# Autodesk Inventor assembly: ASSY,MK4i,Swerve_Module
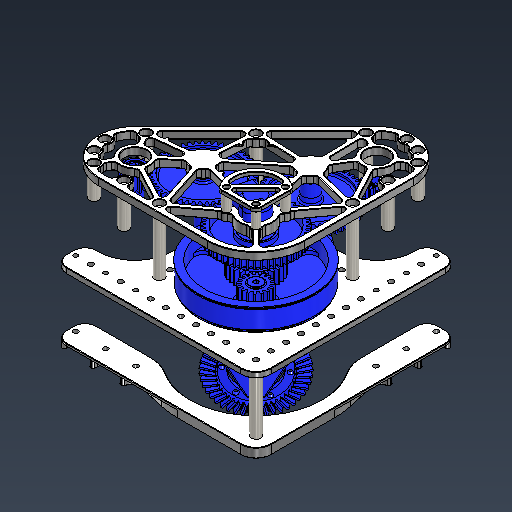
[picture p0: Inventor's stored thumbnail of the model, 512x512]
Saved by Autodesk Inventor 2026 (Build 300175050, 175E)
## iProperties
Created: 2024-01-10
Part Number: ASSY,MK4i,Swerve_Module
Document SubType Name: Assembly
Designer: dave.simone
Mass: 1631.73 g
Surface Area: 2686.09 cm^2
Volume: 361.803 cm^3
Density: 4.51 g/cm^3
Author: dave.simone
## Documents named in this file (9)
- C:\Users\Jthib\Documents\GitHub\2026-Robot-Mechanical\#1_CAD Library\SDS MK4i Swerve\ASSY,MK4i,LOW,Swerve_Module.iam
- C:\Users\Jthib\Documents\GitHub\2026-Robot-Mechanical\#1_CAD Library\SDS MK4i Swerve\PURCHASED_SUB,PLATE,MAIN,MK4i,Swerve.ipt
- C:\Users\Jthib\Documents\GitHub\2026-Robot-Mechanical\#1_CAD Library\SDS MK4i Swerve\PURCHASED_SUB,PLATE,CLAMP,MK4i,Swerve.ipt
- C:\Users\Jthib\Documents\GitHub\2026-Robot-Mechanical\#1_CAD Library\SDS MK4i Swerve\PURCHASED_SUB,PLATE,UPPER,MK4i,Swerve.ipt
- C:\Users\Jthib\Documents\GitHub\2026-Robot-Mechanical\#1_CAD Library\SDS MK4i Swerve\PURCHASED_SUB,PLATE,ENCODER,MK4i,Swerve.ipt
- C:\Users\Jthib\Documents\GitHub\2026-Robot-Mechanical\#1_CAD Library\SDS MK4i Swerve\PURCHASED_SUB,SPACER,SHORT,MK4i,Swerve.ipt
- C:\Users\Jthib\Documents\GitHub\2026-Robot-Mechanical\#1_CAD Library\SDS MK4i Swerve\PURCHASED_SUB,SPACER,LONG,MK4i,Swerve.ipt
- C:\Users\Jthib\Documents\GitHub\2026-Robot-Mechanical\#1_CAD Library\SDS MK4i Swerve\PURCHASED_SUB,SPACER,SHORTER,MK4i,Swerve.ipt
- C:\Users\Jthib\Documents\GitHub\2026-Robot-Mechanical\#1_CAD Library\SDS MK4i Swerve\PURCHASED_SUB,GEAR_TRAIN,WHEEL,MK4i,Swerve.ipt
## Components (18 placed, 8 different names)
1. PURCHASED_SUB,GEAR_TRAIN,WHEEL,MK4i,Swerve:1 — Mate:20, Mate:21
2. PURCHASED_SUB,PLATE,MAIN,MK4i,Swerve:1 — Mate:6, Mate:7, Mate:8, Mate:9, Mate:20, Mate:21, Mate:22, Mate:23, Mate:24, Mate:25, Mate:26
3. PURCHASED_SUB,PLATE,CLAMP,MK4i,Swerve:1 — Mate:22, Mate:23, Mate:24
4. PURCHASED_SUB,PLATE,UPPER,MK4i,Swerve:1 — Insert:4, Insert:5, Insert:6, Insert:7, Insert:8, Insert:9, Insert:10, Insert:11, Insert:12, Insert:20, Insert:21, Insert:22
5. PURCHASED_SUB,SPACER,SHORTER,MK4i,Swerve:1 — Insert:20, Mate:11
6. PURCHASED_SUB,SPACER,SHORTER,MK4i,Swerve:2 — Insert:21, Mate:12
7. PURCHASED_SUB,SPACER,SHORTER,MK4i,Swerve:3 — Insert:22, Mate:13
8. PURCHASED_SUB,SPACER,LONG,MK4i,Swerve:4 — Mate:25, Mate:26
9. PURCHASED_SUB,PLATE,ENCODER,MK4i,Swerve:1 — Mate:11, Mate:12, Mate:13
10. PURCHASED_SUB,SPACER,LONG,MK4i,Swerve:1 — Insert:4, Mate:6, Mate:7
11. PURCHASED_SUB,SPACER,LONG,MK4i,Swerve:2 — Insert:5, Mate:8
12. PURCHASED_SUB,SPACER,LONG,MK4i,Swerve:3 — Insert:6, Mate:9
13. PURCHASED_SUB,SPACER,SHORT,MK4i,Swerve:4 — Insert:8
14. PURCHASED_SUB,SPACER,SHORT,MK4i,Swerve:5 — Insert:7
15. PURCHASED_SUB,SPACER,SHORT,MK4i,Swerve:6 — Insert:9
16. PURCHASED_SUB,SPACER,SHORT,MK4i,Swerve:7 — Insert:10
17. PURCHASED_SUB,SPACER,SHORT,MK4i,Swerve:8 — Insert:11
18. PURCHASED_SUB,SPACER,SHORT,MK4i,Swerve:9 — Insert:12
## Relationships (26: Mate 14, Insert 12)
- Insert:4: PURCHASED_SUB,PLATE,UPPER,MK4i,Swerve:1 ↔ PURCHASED_SUB,SPACER,LONG,MK4i,Swerve:1
- Insert:5: PURCHASED_SUB,PLATE,UPPER,MK4i,Swerve:1 ↔ PURCHASED_SUB,SPACER,LONG,MK4i,Swerve:2
- Insert:6: PURCHASED_SUB,PLATE,UPPER,MK4i,Swerve:1 ↔ PURCHASED_SUB,SPACER,LONG,MK4i,Swerve:3
- Mate:6: PURCHASED_SUB,PLATE,MAIN,MK4i,Swerve:1 ↔ PURCHASED_SUB,SPACER,LONG,MK4i,Swerve:1
- Mate:7: PURCHASED_SUB,PLATE,MAIN,MK4i,Swerve:1 ↔ PURCHASED_SUB,SPACER,LONG,MK4i,Swerve:1
- Mate:8: PURCHASED_SUB,PLATE,MAIN,MK4i,Swerve:1 ↔ PURCHASED_SUB,SPACER,LONG,MK4i,Swerve:2
- Mate:9: PURCHASED_SUB,PLATE,MAIN,MK4i,Swerve:1 ↔ PURCHASED_SUB,SPACER,LONG,MK4i,Swerve:3
- Insert:7: PURCHASED_SUB,PLATE,UPPER,MK4i,Swerve:1 ↔ PURCHASED_SUB,SPACER,SHORT,MK4i,Swerve:5
- Insert:8: PURCHASED_SUB,PLATE,UPPER,MK4i,Swerve:1 ↔ PURCHASED_SUB,SPACER,SHORT,MK4i,Swerve:4
- Insert:9: PURCHASED_SUB,PLATE,UPPER,MK4i,Swerve:1 ↔ PURCHASED_SUB,SPACER,SHORT,MK4i,Swerve:6
- Insert:10: PURCHASED_SUB,PLATE,UPPER,MK4i,Swerve:1 ↔ PURCHASED_SUB,SPACER,SHORT,MK4i,Swerve:7
- Insert:11: PURCHASED_SUB,PLATE,UPPER,MK4i,Swerve:1 ↔ PURCHASED_SUB,SPACER,SHORT,MK4i,Swerve:8
- Insert:12: PURCHASED_SUB,PLATE,UPPER,MK4i,Swerve:1 ↔ PURCHASED_SUB,SPACER,SHORT,MK4i,Swerve:9
- Insert:20: PURCHASED_SUB,PLATE,UPPER,MK4i,Swerve:1 ↔ PURCHASED_SUB,SPACER,SHORTER,MK4i,Swerve:1
- Insert:21: PURCHASED_SUB,PLATE,UPPER,MK4i,Swerve:1 ↔ PURCHASED_SUB,SPACER,SHORTER,MK4i,Swerve:2
- Insert:22: PURCHASED_SUB,PLATE,UPPER,MK4i,Swerve:1 ↔ PURCHASED_SUB,SPACER,SHORTER,MK4i,Swerve:3
- Mate:11: PURCHASED_SUB,SPACER,SHORTER,MK4i,Swerve:1 ↔ PURCHASED_SUB,PLATE,ENCODER,MK4i,Swerve:1
- Mate:12: PURCHASED_SUB,SPACER,SHORTER,MK4i,Swerve:2 ↔ PURCHASED_SUB,PLATE,ENCODER,MK4i,Swerve:1
- Mate:13: PURCHASED_SUB,SPACER,SHORTER,MK4i,Swerve:3 ↔ PURCHASED_SUB,PLATE,ENCODER,MK4i,Swerve:1
- Mate:20: PURCHASED_SUB,GEAR_TRAIN,WHEEL,MK4i,Swerve:1 ↔ PURCHASED_SUB,PLATE,MAIN,MK4i,Swerve:1
- Mate:21: PURCHASED_SUB,GEAR_TRAIN,WHEEL,MK4i,Swerve:1 ↔ PURCHASED_SUB,PLATE,MAIN,MK4i,Swerve:1
- Mate:22: PURCHASED_SUB,PLATE,MAIN,MK4i,Swerve:1 ↔ PURCHASED_SUB,PLATE,CLAMP,MK4i,Swerve:1
- Mate:23: PURCHASED_SUB,PLATE,MAIN,MK4i,Swerve:1 ↔ PURCHASED_SUB,PLATE,CLAMP,MK4i,Swerve:1
- Mate:24 (50.8 mm): PURCHASED_SUB,PLATE,MAIN,MK4i,Swerve:1 ↔ PURCHASED_SUB,PLATE,CLAMP,MK4i,Swerve:1
- Mate:25: PURCHASED_SUB,PLATE,MAIN,MK4i,Swerve:1 ↔ PURCHASED_SUB,SPACER,LONG,MK4i,Swerve:4
- Mate:26: PURCHASED_SUB,PLATE,MAIN,MK4i,Swerve:1 ↔ PURCHASED_SUB,SPACER,LONG,MK4i,Swerve:4
